# Autodesk Inventor assembly: Rasberrypi3case-ver1-1111-2017
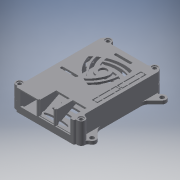
[picture p0: Inventor's stored thumbnail of the model, 180x180]
Saved by Autodesk Inventor 2016 SP1 (Build 200210100, 210)
## iProperties
Created: 2017-02-07
Part Number: Rasberrypi3case-ver1-1111-2017
Document SubType Name: Assembly
Designer: 601898
Author: 601898
## Documents named in this file (3)
- H:\Robotics\GrabCAD\Power Hawks CAD\Electrical Resources\Rasberrypi3case-ver1-1111-2017.iam
- H:\files\rpi2-top.ipt
- H:\files\rpi3-bottom.ipt
## Components (2 placed, 2 different names)
1. rpi2-top:1 — Mate:1, Flush:1, Mate:2
2. rpi3-bottom:1 — Mate:1, Flush:1, Mate:2
## Relationships (3: Mate 2, Flush 1)
- Mate:1: rpi2-top:1 ↔ rpi3-bottom:1
- Flush:1: rpi2-top:1 ↔ rpi3-bottom:1
- Mate:2: rpi2-top:1 ↔ rpi3-bottom:1
